# Autodesk Inventor assembly: am-0801a (-1in) - custom ToughBox Long Hex Shaft with Magnet
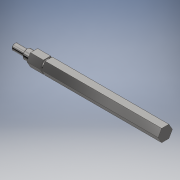
[picture p0: Inventor's stored thumbnail of the model, 180x180]
Saved by Autodesk Inventor 2018 (Build 220112000, 112)
## iProperties
Created: 2018-11-10
Part Number: am-0801a (-1in) - custom ToughBox Long Hex Shaft with Magnet
Document SubType Name: Weldment
Designer: TODD D MILLER
Weld Material: Welded Aluminum-6061
Author: TODD D MILLER
## Documents named in this file (2)
- G:\FRC\CAD Library\SHAFTS\am-0801a (-1in) - custom ToughBox Long Hex Shaft with Magnet.iam
- G:\FRC\CAD Library\SHAFTS\am-0801a - Toughbox Long Hex Shaft with Magnet.ipt
## Components (1 placed, 1 different names)
1. am-0801a - Toughbox Long Hex Shaft with Magnet:1
## Named parameters: cut_length = 25.4 mm
